# Autodesk Inventor assembly: Zespół1
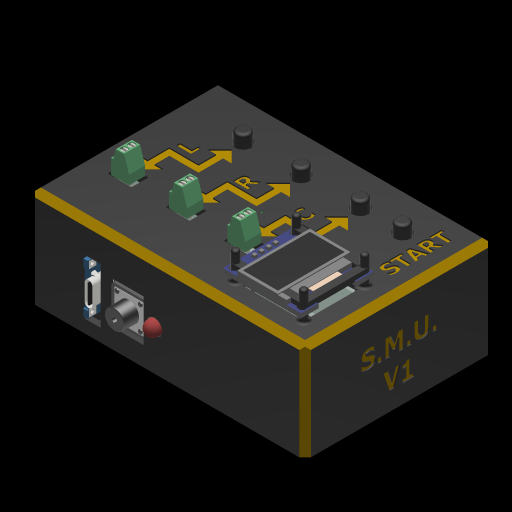
[picture p0: Inventor's stored thumbnail of the model, 512x512]
Saved by Autodesk Inventor 2024.4 (Build 284460000, 460)
## iProperties
Created: 2026-01-14
Part Number: Zespół1
Document SubType Name: Assembly
Designer: User
Author: User
## iProperties of the stored document 5mm_LED_Red.ipt
Created: 2026-01-16
Part Number: 5mm_LED_Red
Material: Generic
Document SubType Name: Modeling
Designer: rk
Mass: 0.169759 g
Surface Area: 2.48677 cm^2
Volume: 0.169759 cm^3
Density: 1 g/cm^3
Appearance: Domyślna
Sending System: Autodesk Inventor 2025
Author: rk
Revision Number: 0
## Documents named in this file (13)
- C:\Users\Duszy\Desktop\Projekty\S.M.T\Obudowa\Zespół1.iam
- C:\Users\Duszy\Downloads\raspberry-pi-pico-w-2.snapshot.8\Raspberry_Pi_Pico_W.ipt
- C:\Users\Duszy\Desktop\Projekty\S.M.T\Miernik\Miernik.ipt
- C:\Users\Duszy\Desktop\Projekty\S.M.T\Obudowa\spod.ipt
- C:\Users\Duszy\Desktop\Projekty\S.M.T\Obudowa\atrapa_ogniwa.ipt
- C:\Users\Duszy\Desktop\Projekty\S.M.T\Obudowa\gora.ipt
- C:\Users\Duszy\Downloads\0-9-inch-i2c-oled-128x64-display-module-1.snapshot.1\0.9 inch I2C OLED 128×64 Display Module_jhalak.ipt
- C:\Users\Duszy\Desktop\Projekty\S.M.T\Obudowa\button.ipt
- C:\Users\Duszy\Desktop\Projekty\S.M.T\Obudowa\TerminalBlock_Phoenix_MPT-0,5-2-2.54_1x02_P2.54mm_Horizontal\TerminalBlock_Phoenix_MPT-0,5-2-2.54_1x02_P2.54mm_Horizontal\TerminalBlock_Phoenix_MPT-0,5-2-2.54_1x02_.ipt
- **C:\Users\Duszy\Desktop\Projekty\S.M.T\Obudowa\Zespół1.iam*LocalDocs*xAaaaa5caAaaaaaaaAaaaq10vPe*5mm_LED_Red.ipt
- C:\Users\Duszy\Desktop\Projekty\S.M.T\Obudowa\TP4056_Charging_Module_Type_C\TP4056_Charging_Module_Type_C\TP4056_Charging_Module_Type_C.ipt
- C:\Users\Duszy\Desktop\Projekty\S.M.T\Obudowa\12x12x8mm\12x12x8mm\12x12x8mm.ipt
- C:\Users\Duszy\Desktop\Projekty\S.M.T\Obudowa\5mm_LED_Red.ipt
## Components (16 placed, 11 different names)
1. Miernik:1 — Obrotowe:2
2. spod:1 — Obrotowe:1, Obrotowe:2, Sztywne:4, Sztywne:6, Sztywne:7, Sztywne:8
3. Raspberry_Pi_Pico_W:1 — Obrotowe:1
4. atrapa_ogniwa:1
5. gora:1 — Sztywne:4, Sztywne:5, Obrotowe:3, Sztywne:9
6. 0.9 inch I2C OLED 128×64 Display Module_jhalak:1
7. 5mm_LED_Red:1 — Sztywne:6
8. TP4056_Charging_Module_Type_C:1 — Sztywne:7
9. 12x12x8mm:1 — Sztywne:8
10. button:2 — Sztywne:5
11. button:3
12. button:4 — Obrotowe:3
13. button:5
14. TerminalBlock_Phoenix_MPT-0,5-2-2.54_1x02_:1 — Sztywne:9
15. TerminalBlock_Phoenix_MPT-0,5-2-2.54_1x02_:2
16. TerminalBlock_Phoenix_MPT-0,5-2-2.54_1x02_:3
## Component patterns: (2 elements, first: button:2), (2 elements, first: button:4), (3 elements, first: TerminalBlock_Phoenix_MPT-0,5-2-2.54_1x02_:1)
## Relationships (9: WeldJoint 6, RevoluteJoint 3)
- Obrotowe:1 [RevoluteJoint] (-5 mm): spod:1 ↔ Raspberry_Pi_Pico_W:1
- Obrotowe:2 [RevoluteJoint] (-1 mm): Miernik:1 ↔ spod:1
- Sztywne:4 [WeldJoint] (1 mm): spod:1 ↔ gora:1
- Sztywne:5 [WeldJoint]: gora:1 ↔ button:2
- Obrotowe:3 [RevoluteJoint] (-1.3 mm): gora:1 ↔ button:4
- Sztywne:6 [WeldJoint]: spod:1 ↔ 5mm_LED_Red:1
- Sztywne:7 [WeldJoint]: spod:1 ↔ TP4056_Charging_Module_Type_C:1
- Sztywne:8 [WeldJoint]: spod:1 ↔ 12x12x8mm:1
- Sztywne:9 [WeldJoint] (1 mm): gora:1 ↔ TerminalBlock_Phoenix_MPT-0,5-2-2.54_1x02_:1
